# Autodesk Inventor assembly: Assemlby_OpenOxygen
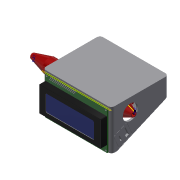
[picture p0: Inventor's stored thumbnail of the model, 180x180]
Saved by Autodesk Inventor 2019.4 (Build 234330000, 330)
## iProperties
Created: 2021-06-01
Part Number: Assemlby_OpenOxygen
Document SubType Name: Assembly
Designer: diederichbenedict
Author: diederichbenedict
## Documents named in this file (10)
- C:\Users\diederichbenedict\Dropbox\Dokumente\Promotion\PROJECTS\OXYGEN\INVENTOR\Assemlby_OpenOxygen.iam
- C:\Users\diederichbenedict\Dropbox\Dokumente\Promotion\PROJECTS\OXYGEN\INVENTOR\00_Sensirion_Flowsensor.ipt
- C:\Users\diederichbenedict\Dropbox\Dokumente\Promotion\PROJECTS\OXYGEN\INVENTOR\00_Arduino_LCD_I2Cstep.ipt
- C:\Users\diederichbenedict\Dropbox\Dokumente\Promotion\PROJECTS\OXYGEN\INVENTOR\00_ESP32.ipt
- C:\Users\diederichbenedict\Dropbox\Dokumente\Promotion\PROJECTS\OXYGEN\INVENTOR\00_Oxygen_Oxi.ipt
- C:\Users\diederichbenedict\Dropbox\Dokumente\Promotion\PROJECTS\OXYGEN\INVENTOR\00_LM286.ipt
- C:\Users\diederichbenedict\Dropbox\Dokumente\Promotion\PROJECTS\OXYGEN\INVENTOR\01_Connector_T.ipt
- C:\Users\diederichbenedict\Dropbox\Dokumente\Promotion\PROJECTS\OXYGEN\INVENTOR\02_Connector_S.ipt
- C:\Users\diederichbenedict\Dropbox\Dokumente\Promotion\PROJECTS\OXYGEN\INVENTOR\03_OpenOxygen_Box.ipt
- C:\Users\diederichbenedict\Dropbox\Dokumente\Promotion\PROJECTS\OXYGEN\INVENTOR\00_Batterypack.ipt
## Components (9 placed, 9 different names)
1. 00_Sensirion_Flowsensor:1 — Flush:1, Angle:1, Flush:2, Flush:4, Insert:1, Insert:3
2. 00_Arduino_LCD_I2Cstep:1 — Flush:1, Angle:1, Flush:2, Flush:5, Flush:6
3. 00_LM286:1 — Flush:4
4. 01_Connector_T:1 — Insert:1, Insert:2
5. 00_Oxygen_Oxi:1 — Insert:2
6. 02_Connector_S:1 — Insert:3
7. 03_OpenOxygen_Box:1 — Flush:5, Flush:6, Angle:4, Flush:7, Flush:8, Mate:1
8. 00_Batterypack:1 — Angle:4, Flush:7, Flush:8, Mate:1
9. 00_ESP32:1
## Relationships (13: Flush 7, Insert 3, Angle 2, Mate 1)
- Flush:1 (5 mm): 00_Sensirion_Flowsensor:1 ↔ 00_Arduino_LCD_I2Cstep:1
- Angle:1 (180 deg): 00_Sensirion_Flowsensor:1 ↔ 00_Arduino_LCD_I2Cstep:1
- Flush:2 (-10 mm): 00_Sensirion_Flowsensor:1 ↔ 00_Arduino_LCD_I2Cstep:1
- Flush:4: 00_Sensirion_Flowsensor:1 ↔ 00_LM286:1
- Insert:1: 00_Sensirion_Flowsensor:1 ↔ 01_Connector_T:1
- Insert:2: 01_Connector_T:1 ↔ 00_Oxygen_Oxi:1
- Insert:3: 00_Sensirion_Flowsensor:1 ↔ 02_Connector_S:1
- Flush:5: 00_Arduino_LCD_I2Cstep:1 ↔ 03_OpenOxygen_Box:1
- Flush:6: 00_Arduino_LCD_I2Cstep:1 ↔ 03_OpenOxygen_Box:1
- Angle:4 (0 deg): 03_OpenOxygen_Box:1 ↔ 00_Batterypack:1
- Flush:7: 03_OpenOxygen_Box:1 ↔ 00_Batterypack:1
- Flush:8 (1 mm): 03_OpenOxygen_Box:1 ↔ 00_Batterypack:1
- Mate:1 (4 mm): 03_OpenOxygen_Box:1 ↔ 00_Batterypack:1
